# Autodesk Inventor assembly: Custom_Delta_Assembly
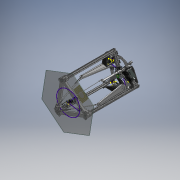
[picture p0: Inventor's stored thumbnail of the model, 180x180]
Saved by Autodesk Inventor 2019.4 (Build 234330000, 330)
## iProperties
Created: 2019-07-06
Part Number: Custom_Delta_Assembly
Document SubType Name: Assembly
Designer: Jorian Brusind
Author: Jorian Brusind
## Documents named in this file (20)
- C:\Users\Jorian Bruslind\Documents\GitHub\ECE44x_Senior_Design\Design files\Delta Robot Arm\Inventor Files\Custom_Delta\Custom_Delta_Assembly.iam
- C:\Users\Jorian Bruslind\Documents\GitHub\ECE44x_Senior_Design\Design files\Delta Robot Arm\Inventor Files\Custom_Delta\Stepper_Face.ipt
- C:\Users\Jorian Bruslind\Documents\GitHub\ECE44x_Senior_Design\Design files\Delta Robot Arm\Inventor Files\Custom_Delta\Delta_Arm.ipt
- C:\Users\Jorian Bruslind\Documents\GitHub\ECE44x_Senior_Design\Design files\Delta Robot Arm\Inventor Files\Custom_Delta\Delta_Top.ipt
- C:\Users\Jorian Bruslind\Documents\GitHub\ECE44x_Senior_Design\Design files\Delta Robot Arm\Inventor Files\McMaster Files\59935K140_METRIC BALL JOINT ROD END.ipt
- C:\Users\Jorian Bruslind\Documents\GitHub\ECE44x_Senior_Design\Design files\PetriFilm\PetriFilm.iam
- C:\Users\Jorian Bruslind\Documents\GitHub\ECE44x_Senior_Design\Design files\Delta Robot Arm\Inventor Files\McMaster Files\5537T501_ALUMINUM T-SLOTTED FRAMING EXTRUSION.ipt
- C:\Users\Jorian Bruslind\Documents\GitHub\ECE44x_Senior_Design\Design files\Delta Robot Arm\Inventor Files\McMaster Files\5537T518_T-SLOTTED FRAMING.ipt
- C:\Users\Jorian Bruslind\Documents\GitHub\ECE44x_Senior_Design\Design files\Delta Robot Arm\Inventor Files\McMaster Files\6In_ALUMINUM T-SLOTTED FRAMING EXTRUSION.ipt
- C:\Users\Jorian Bruslind\Documents\GitHub\ECE44x_Senior_Design\Design files\Delta Robot Arm\Inventor Files\Custom_Delta\Custom_Delta_End_Effector.ipt
- C:\Users\Jorian Bruslind\Documents\GitHub\ECE44x_Senior_Design\Design files\Delta Robot Arm\Inventor Files\Custom_Delta\80_20_Connector.ipt
- C:\Users\Jorian Bruslind\Documents\GitHub\ECE44x_Senior_Design\Design files\Delta Robot Arm\Inventor Files\Custom_Delta\NEMA17_Stepper_CL42H60.ipt
- C:\Users\Jorian Bruslind\Documents\GitHub\ECE44x_Senior_Design\Design files\Delta Robot Arm\Inventor Files\Stepper_Collar\products\12196\step\model.ipt
- C:\Users\Jorian Bruslind\Documents\GitHub\ECE44x_Senior_Design\Design files\Delta Robot Arm\Inventor Files\raspberry-pi-camera-module-v2-1.snapshot.3\RspCameraMia.iam
- C:\Users\Jorian Bruslind\Documents\GitHub\ECE44x_Senior_Design\Design files\Delta Robot Arm\Inventor Files\Custom_Delta\80_20_Connector_Bot.ipt
- C:\Users\Jorian Bruslind\Documents\GitHub\ECE44x_Senior_Design\Design files\Delta Robot Arm\Inventor Files\endstop-mechanical-limit-switch-on-pcb-1.snapshot.1\Switch.ipt
- C:\Users\Jorian Bruslind\Documents\GitHub\ECE44x_Senior_Design\Design files\Delta Robot Arm\Inventor Files\Metric bolt\Bolt M3 30mm.ipt
- C:\Users\Jorian Bruslind\Documents\GitHub\ECE44x_Senior_Design\Design files\Delta Robot Arm\Inventor Files\Custom_Delta\5mmSpacer.ipt
- C:\Users\Jorian Bruslind\Documents\GitHub\ECE44x_Senior_Design\Design files\Delta Robot Arm\Inventor Files\Custom_Delta\Bottom_Mount.ipt
- C:\Users\Jorian Bruslind\Documents\GitHub\ECE44x_Senior_Design\Design files\Delta Robot Arm\Inventor Files\McMaster Files\98861A050_LOW-STRENGTH STEEL THREADED ROD.ipt
## Components (60 placed, 19 different names)
1. Stepper_Face:1 — Mate:126, Flush:20, Flush:23, Mate:210, Mate:211, Mate:212, Mate:216
2. Delta_Arm:1 — Mate:145, Mate:146, Mate:214, Mate:215, Mate:254, Mate:360, Mate:361
3. Stepper_Face:2 — Mate:125, Flush:18, Flush:24, Mate:222, Mate:227, Mate:230, Mate:231
4. Delta_Arm:2 — Mate:151, Mate:152, Mate:220, Mate:221, Mate:253, Mate:321
5. Stepper_Face:3 — Mate:127, Flush:21, Flush:22, Mate:217, Mate:218, Mate:226, Mate:228
6. Delta_Arm:3 — Mate:224, Mate:225, Mate:229, Mate:333, Mate:341, Mate:345, Mate:346
7. Delta_Top:1 — Mate:103, Mate:105, Mate:106, Mate:107, Mate:109, Mate:110, Mate:111, Mate:112, Mate:113, Mate:189, Mate:190, Mate:191, Mate:192, Mate:238, Mate:240, Mate:241, Mate:243, Mate:244, Mate:246, Mate:368
8. 59935K140_METRIC BALL JOINT ROD END:2 — Mate:145, Mate:146
9. 59935K140_METRIC BALL JOINT ROD END:3 — Mate:151, Mate:152, Mate:270, Mate:271, Mate:374
10. PetriFilm:1 [sub-assembly]
11. 5537T518_T-SLOTTED FRAMING:1 — Mate:106, Mate:107, Mate:119, Flush:30
12. 5537T518_T-SLOTTED FRAMING:2 — Mate:103, Mate:105, Mate:118
13. 5537T518_T-SLOTTED FRAMING:3 — Mate:109, Mate:110, Mate:117
14. 6In_ALUMINUM T-SLOTTED FRAMING EXTRUSION:1 — Flush:5, Mate:121, Flush:6, Mate:126, Flush:20, Flush:23, Mate:188, Mate:235, Mate:247
15. 6In_ALUMINUM T-SLOTTED FRAMING EXTRUSION:2 — Flush:9, Flush:10, Mate:123, Mate:125, Flush:18, Flush:24, Mate:237
16. 6In_ALUMINUM T-SLOTTED FRAMING EXTRUSION:3 — Flush:7, Flush:8, Mate:122, Mate:127, Flush:21, Flush:22, Mate:233
17. 5537T501_ALUMINUM T-SLOTTED FRAMING EXTRUSION:1 — Mate:112, Mate:118, Flush:5, Mate:121, Flush:6, Mate:192, Mate:234, Flush:26, Mate:245, Mate:357, Mate:358
18. 5537T501_ALUMINUM T-SLOTTED FRAMING EXTRUSION:2 — Mate:111, Mate:119, Flush:7, Flush:8, Mate:122, Mate:190, Mate:232, Flush:25, Mate:239, Mate:355, Mate:359
19. 5537T501_ALUMINUM T-SLOTTED FRAMING EXTRUSION:3 — Mate:113, Mate:117, Flush:9, Flush:10, Mate:123, Mate:191, Mate:236, Flush:27, Mate:242, Mate:354, Mate:356
20. 80_20_Connector:1 — Mate:188, Mate:189, Mate:248, Mate:249, Mate:255, Mate:256, Mate:263, Mate:264, Mate:265, Mate:266, Mate:267
21. NEMA17_Stepper_CL42H60:1 — Mate:219, Mate:227, Mate:230, Mate:231
22. NEMA17_Stepper_CL42H60:2 — Mate:210, Mate:211, Mate:212, Mate:213
23. NEMA17_Stepper_CL42H60:3 — Mate:217, Mate:218, Mate:223, Mate:228
24. model:4 — Mate:223, Mate:224, Mate:225, Mate:226, Mate:229
25. model:5 — Mate:213, Mate:214, Mate:215, Mate:216, Mate:254
26. model:6 — Mate:219, Mate:220, Mate:221, Mate:222, Mate:253
27. 5537T518_T-SLOTTED FRAMING:4 — Mate:236, Mate:237, Flush:27
28. 5537T518_T-SLOTTED FRAMING:5 — Mate:232, Mate:233, Flush:25
29. 5537T518_T-SLOTTED FRAMING:6 — Mate:234, Mate:235, Flush:26
30. 5537T518_T-SLOTTED FRAMING:7 — Mate:238, Mate:239, Mate:240, Flush:28
31. 5537T518_T-SLOTTED FRAMING:8 — Mate:241, Mate:242, Mate:243
32. 5537T518_T-SLOTTED FRAMING:9 — Mate:244, Mate:245, Mate:246, Flush:29
33. RspCameraMia:1 [sub-assembly] — Mate:250, Mate:251, Mate:252
34. 80_20_Connector_Bot:1 — Mate:247, Mate:248, Mate:249, Mate:250, Mate:251, Mate:252
35. Switch:1 — Mate:255, Mate:256, Mate:263
36. Switch:2
37. Switch:3
38. 80_20_Connector:2 — Mate:264, Mate:265, Mate:266, Mate:268, Mate:269
39. 80_20_Connector:3 — Mate:267, Mate:268, Mate:269
40. Bolt M3 30mm:1 — Mate:270, Mate:271, Mate:299, Mate:320
41. 5mmSpacer:2 — Mate:299
42. 59935K140_METRIC BALL JOINT ROD END:17 — Mate:320, Mate:321, Mate:370, Mate:372
43. 59935K140_METRIC BALL JOINT ROD END:22 — Mate:333, Mate:346, Mate:380, Mate:382
44. 59935K140_METRIC BALL JOINT ROD END:23 — Mate:341, Mate:345, Mate:377, Mate:379
45. Bottom_Mount:1 — Mate:354, Mate:355, Flush:28
46. Bottom_Mount:3 — Mate:356, Mate:357, Flush:29
47. Bottom_Mount:4 — Mate:358, Mate:359, Flush:30
48. 59935K140_METRIC BALL JOINT ROD END:24 — Mate:360, Mate:361, Mate:385, Mate:386
49. 98861A050_LOW-STRENGTH STEEL THREADED ROD:2 — Mate:369, Mate:370, Mate:371, Mate:372
50. 98861A050_LOW-STRENGTH STEEL THREADED ROD:3 — Mate:376, Mate:377, Mate:378, Mate:379
51. 98861A050_LOW-STRENGTH STEEL THREADED ROD:4 — Mate:380, Mate:382, Mate:383
52. 98861A050_LOW-STRENGTH STEEL THREADED ROD:5 — Mate:373, Mate:374, Mate:375
53. 98861A050_LOW-STRENGTH STEEL THREADED ROD:6 — Mate:384, Mate:385, Mate:386, Mate:387
54. 59935K140_METRIC BALL JOINT ROD END:25 — Mate:364, Mate:376, Mate:378
55. 59935K140_METRIC BALL JOINT ROD END:26 — Mate:363, Mate:369, Mate:371
56. 59935K140_METRIC BALL JOINT ROD END:27 — Mate:366, Mate:384, Mate:387
57. 59935K140_METRIC BALL JOINT ROD END:28 — Mate:362, Mate:373, Mate:375
58. 59935K140_METRIC BALL JOINT ROD END:29 — Mate:367
59. 59935K140_METRIC BALL JOINT ROD END:30 — Mate:365, Mate:383
60. Custom_Delta_End_Effector:1 — Mate:362, Mate:363, Mate:364, Mate:365, Mate:366, Mate:367, Mate:368
## Relationships (141: Mate 123, Flush 18)
- Mate:103: Delta_Top:1 ↔ 5537T518_T-SLOTTED FRAMING:2
- Mate:105: Delta_Top:1 ↔ 5537T518_T-SLOTTED FRAMING:2
- Mate:106: Delta_Top:1 ↔ 5537T518_T-SLOTTED FRAMING:1
- Mate:107: Delta_Top:1 ↔ 5537T518_T-SLOTTED FRAMING:1
- Mate:109: Delta_Top:1 ↔ 5537T518_T-SLOTTED FRAMING:3
- Mate:110: Delta_Top:1 ↔ 5537T518_T-SLOTTED FRAMING:3
- Mate:111: Delta_Top:1 ↔ 5537T501_ALUMINUM T-SLOTTED FRAMING EXTRUSION:2
- Mate:112: Delta_Top:1 ↔ 5537T501_ALUMINUM T-SLOTTED FRAMING EXTRUSION:1
- Mate:113: Delta_Top:1 ↔ 5537T501_ALUMINUM T-SLOTTED FRAMING EXTRUSION:3
- Mate:117: 5537T518_T-SLOTTED FRAMING:3 ↔ 5537T501_ALUMINUM T-SLOTTED FRAMING EXTRUSION:3
- Mate:118: 5537T518_T-SLOTTED FRAMING:2 ↔ 5537T501_ALUMINUM T-SLOTTED FRAMING EXTRUSION:1
- Mate:119: 5537T518_T-SLOTTED FRAMING:1 ↔ 5537T501_ALUMINUM T-SLOTTED FRAMING EXTRUSION:2
- Flush:5: 6In_ALUMINUM T-SLOTTED FRAMING EXTRUSION:1 ↔ 5537T501_ALUMINUM T-SLOTTED FRAMING EXTRUSION:1
- Mate:121: 6In_ALUMINUM T-SLOTTED FRAMING EXTRUSION:1 ↔ 5537T501_ALUMINUM T-SLOTTED FRAMING EXTRUSION:1
- Flush:6: 6In_ALUMINUM T-SLOTTED FRAMING EXTRUSION:1 ↔ 5537T501_ALUMINUM T-SLOTTED FRAMING EXTRUSION:1
- Flush:7: 6In_ALUMINUM T-SLOTTED FRAMING EXTRUSION:3 ↔ 5537T501_ALUMINUM T-SLOTTED FRAMING EXTRUSION:2
- Flush:8: 6In_ALUMINUM T-SLOTTED FRAMING EXTRUSION:3 ↔ 5537T501_ALUMINUM T-SLOTTED FRAMING EXTRUSION:2
- Mate:122: 6In_ALUMINUM T-SLOTTED FRAMING EXTRUSION:3 ↔ 5537T501_ALUMINUM T-SLOTTED FRAMING EXTRUSION:2
- Flush:9: 6In_ALUMINUM T-SLOTTED FRAMING EXTRUSION:2 ↔ 5537T501_ALUMINUM T-SLOTTED FRAMING EXTRUSION:3
- Flush:10: 6In_ALUMINUM T-SLOTTED FRAMING EXTRUSION:2 ↔ 5537T501_ALUMINUM T-SLOTTED FRAMING EXTRUSION:3
- Mate:123: 6In_ALUMINUM T-SLOTTED FRAMING EXTRUSION:2 ↔ 5537T501_ALUMINUM T-SLOTTED FRAMING EXTRUSION:3
- Mate:125: Stepper_Face:2 ↔ 6In_ALUMINUM T-SLOTTED FRAMING EXTRUSION:2
- Mate:126: Stepper_Face:1 ↔ 6In_ALUMINUM T-SLOTTED FRAMING EXTRUSION:1
- Mate:127: Stepper_Face:3 ↔ 6In_ALUMINUM T-SLOTTED FRAMING EXTRUSION:3
- Mate:145: Delta_Arm:1 ↔ 59935K140_METRIC BALL JOINT ROD END:2
- Mate:146 (2.5 mm): Delta_Arm:1 ↔ 59935K140_METRIC BALL JOINT ROD END:2
- Mate:151: Delta_Arm:2 ↔ 59935K140_METRIC BALL JOINT ROD END:3
- Mate:152 (2.5 mm): Delta_Arm:2 ↔ 59935K140_METRIC BALL JOINT ROD END:3
- Flush:18: Stepper_Face:2 ↔ 6In_ALUMINUM T-SLOTTED FRAMING EXTRUSION:2
- Flush:20: Stepper_Face:1 ↔ 6In_ALUMINUM T-SLOTTED FRAMING EXTRUSION:1
- Flush:21: Stepper_Face:3 ↔ 6In_ALUMINUM T-SLOTTED FRAMING EXTRUSION:3
- Flush:22 (112.406 mm): Stepper_Face:3 ↔ 6In_ALUMINUM T-SLOTTED FRAMING EXTRUSION:3
- Flush:23 (112.206 mm): Stepper_Face:1 ↔ 6In_ALUMINUM T-SLOTTED FRAMING EXTRUSION:1
- Flush:24 (112.406 mm): Stepper_Face:2 ↔ 6In_ALUMINUM T-SLOTTED FRAMING EXTRUSION:2
- Mate:188: 6In_ALUMINUM T-SLOTTED FRAMING EXTRUSION:1 ↔ 80_20_Connector:1
- Mate:189: Delta_Top:1 ↔ 80_20_Connector:1
- Mate:190: Delta_Top:1 ↔ 5537T501_ALUMINUM T-SLOTTED FRAMING EXTRUSION:2
- Mate:191: Delta_Top:1 ↔ 5537T501_ALUMINUM T-SLOTTED FRAMING EXTRUSION:3
- Mate:192: Delta_Top:1 ↔ 5537T501_ALUMINUM T-SLOTTED FRAMING EXTRUSION:1
- Mate:210: Stepper_Face:1 ↔ NEMA17_Stepper_CL42H60:2
- Mate:211: Stepper_Face:1 ↔ NEMA17_Stepper_CL42H60:2
- Mate:212: Stepper_Face:1 ↔ NEMA17_Stepper_CL42H60:2
- Mate:213: NEMA17_Stepper_CL42H60:2 ↔ model:5
- Mate:214: Delta_Arm:1 ↔ model:5
- Mate:215: Delta_Arm:1 ↔ model:5
- Mate:216: Stepper_Face:1 ↔ model:5
- Mate:217: Stepper_Face:3 ↔ NEMA17_Stepper_CL42H60:3
- Mate:218: Stepper_Face:3 ↔ NEMA17_Stepper_CL42H60:3
- Mate:219: NEMA17_Stepper_CL42H60:1 ↔ model:6
- Mate:220: Delta_Arm:2 ↔ model:6
- Mate:221: Delta_Arm:2 ↔ model:6
- Mate:222: Stepper_Face:2 ↔ model:6
- Mate:223: NEMA17_Stepper_CL42H60:3 ↔ model:4
- Mate:224: Delta_Arm:3 ↔ model:4
- Mate:225: Delta_Arm:3 ↔ model:4
- Mate:226: Stepper_Face:3 ↔ model:4
- Mate:227: Stepper_Face:2 ↔ NEMA17_Stepper_CL42H60:1
- Mate:228: Stepper_Face:3 ↔ NEMA17_Stepper_CL42H60:3
- Mate:229: Delta_Arm:3 ↔ model:4
- Mate:230: Stepper_Face:2 ↔ NEMA17_Stepper_CL42H60:1
- Mate:231: Stepper_Face:2 ↔ NEMA17_Stepper_CL42H60:1
- Mate:232: 5537T501_ALUMINUM T-SLOTTED FRAMING EXTRUSION:2 ↔ 5537T518_T-SLOTTED FRAMING:5
- Mate:233: 6In_ALUMINUM T-SLOTTED FRAMING EXTRUSION:3 ↔ 5537T518_T-SLOTTED FRAMING:5
- Flush:25: 5537T501_ALUMINUM T-SLOTTED FRAMING EXTRUSION:2 ↔ 5537T518_T-SLOTTED FRAMING:5
- Mate:234: 5537T501_ALUMINUM T-SLOTTED FRAMING EXTRUSION:1 ↔ 5537T518_T-SLOTTED FRAMING:6
- Mate:235: 6In_ALUMINUM T-SLOTTED FRAMING EXTRUSION:1 ↔ 5537T518_T-SLOTTED FRAMING:6
- Flush:26: 5537T501_ALUMINUM T-SLOTTED FRAMING EXTRUSION:1 ↔ 5537T518_T-SLOTTED FRAMING:6
- Mate:236: 5537T501_ALUMINUM T-SLOTTED FRAMING EXTRUSION:3 ↔ 5537T518_T-SLOTTED FRAMING:4
- Mate:237: 6In_ALUMINUM T-SLOTTED FRAMING EXTRUSION:2 ↔ 5537T518_T-SLOTTED FRAMING:4
- Flush:27: 5537T501_ALUMINUM T-SLOTTED FRAMING EXTRUSION:3 ↔ 5537T518_T-SLOTTED FRAMING:4
- Mate:238: Delta_Top:1 ↔ 5537T518_T-SLOTTED FRAMING:7
- Mate:239: 5537T501_ALUMINUM T-SLOTTED FRAMING EXTRUSION:2 ↔ 5537T518_T-SLOTTED FRAMING:7
- Mate:240: Delta_Top:1 ↔ 5537T518_T-SLOTTED FRAMING:7
- Mate:241: Delta_Top:1 ↔ 5537T518_T-SLOTTED FRAMING:8
- Mate:242: 5537T501_ALUMINUM T-SLOTTED FRAMING EXTRUSION:3 ↔ 5537T518_T-SLOTTED FRAMING:8
- Mate:243: Delta_Top:1 ↔ 5537T518_T-SLOTTED FRAMING:8
- Mate:244: Delta_Top:1 ↔ 5537T518_T-SLOTTED FRAMING:9
- Mate:245: 5537T501_ALUMINUM T-SLOTTED FRAMING EXTRUSION:1 ↔ 5537T518_T-SLOTTED FRAMING:9
- Mate:246: Delta_Top:1 ↔ 5537T518_T-SLOTTED FRAMING:9
- Mate:247: 6In_ALUMINUM T-SLOTTED FRAMING EXTRUSION:1 ↔ 80_20_Connector_Bot:1
- Mate:248: 80_20_Connector:1 ↔ 80_20_Connector_Bot:1
- Mate:249: 80_20_Connector:1 ↔ 80_20_Connector_Bot:1
- Mate:250: RspCameraMia:1 ↔ 80_20_Connector_Bot:1
- Mate:251: RspCameraMia:1 ↔ 80_20_Connector_Bot:1
- Mate:252: RspCameraMia:1 ↔ 80_20_Connector_Bot:1
- Mate:253: Delta_Arm:2 ↔ model:6
- Mate:254: Delta_Arm:1 ↔ model:5
- Mate:255: 80_20_Connector:1 ↔ Switch:1
- Mate:256: 80_20_Connector:1 ↔ Switch:1
- Mate:263: 80_20_Connector:1 ↔ Switch:1
- Mate:264: 80_20_Connector:1 ↔ 80_20_Connector:2
- Mate:265: 80_20_Connector:1 ↔ 80_20_Connector:2
- Mate:266: 80_20_Connector:1 ↔ 80_20_Connector:2
- Mate:267: 80_20_Connector:1 ↔ 80_20_Connector:3
- Mate:268: 80_20_Connector:2 ↔ 80_20_Connector:3
- Mate:269: 80_20_Connector:2 ↔ 80_20_Connector:3
- Mate:270: 59935K140_METRIC BALL JOINT ROD END:3 ↔ Bolt M3 30mm:1
- Mate:271: 59935K140_METRIC BALL JOINT ROD END:3 ↔ Bolt M3 30mm:1
- Mate:299: Bolt M3 30mm:1 ↔ 5mmSpacer:2
- Mate:320: Bolt M3 30mm:1 ↔ 59935K140_METRIC BALL JOINT ROD END:17
- Mate:321 (2.5 mm): Delta_Arm:2 ↔ 59935K140_METRIC BALL JOINT ROD END:17
- Mate:333: Delta_Arm:3 ↔ 59935K140_METRIC BALL JOINT ROD END:22
- Mate:341: Delta_Arm:3 ↔ 59935K140_METRIC BALL JOINT ROD END:23
- Mate:345 (2.5 mm): Delta_Arm:3 ↔ 59935K140_METRIC BALL JOINT ROD END:23
- Mate:346 (2.5 mm): Delta_Arm:3 ↔ 59935K140_METRIC BALL JOINT ROD END:22
- Mate:354: 5537T501_ALUMINUM T-SLOTTED FRAMING EXTRUSION:3 ↔ Bottom_Mount:1
- Mate:355: 5537T501_ALUMINUM T-SLOTTED FRAMING EXTRUSION:2 ↔ Bottom_Mount:1
- Flush:28: 5537T518_T-SLOTTED FRAMING:7 ↔ Bottom_Mount:1
- Mate:356: 5537T501_ALUMINUM T-SLOTTED FRAMING EXTRUSION:3 ↔ Bottom_Mount:3
- Mate:357: 5537T501_ALUMINUM T-SLOTTED FRAMING EXTRUSION:1 ↔ Bottom_Mount:3
- Flush:29: 5537T518_T-SLOTTED FRAMING:9 ↔ Bottom_Mount:3
- Mate:358: 5537T501_ALUMINUM T-SLOTTED FRAMING EXTRUSION:1 ↔ Bottom_Mount:4
- Mate:359: 5537T501_ALUMINUM T-SLOTTED FRAMING EXTRUSION:2 ↔ Bottom_Mount:4
- Flush:30: 5537T518_T-SLOTTED FRAMING:1 ↔ Bottom_Mount:4
- Mate:360: Delta_Arm:1 ↔ 59935K140_METRIC BALL JOINT ROD END:24
- Mate:361 (2.5 mm): Delta_Arm:1 ↔ 59935K140_METRIC BALL JOINT ROD END:24
- Mate:362: 59935K140_METRIC BALL JOINT ROD END:28 ↔ Custom_Delta_End_Effector:1
- Mate:363: 59935K140_METRIC BALL JOINT ROD END:26 ↔ Custom_Delta_End_Effector:1
- Mate:364: 59935K140_METRIC BALL JOINT ROD END:25 ↔ Custom_Delta_End_Effector:1
- Mate:365: 59935K140_METRIC BALL JOINT ROD END:30 ↔ Custom_Delta_End_Effector:1
- Mate:366: 59935K140_METRIC BALL JOINT ROD END:27 ↔ Custom_Delta_End_Effector:1
- Mate:367: 59935K140_METRIC BALL JOINT ROD END:29 ↔ Custom_Delta_End_Effector:1
- Mate:368: Delta_Top:1 ↔ Custom_Delta_End_Effector:1
- Mate:369: 98861A050_LOW-STRENGTH STEEL THREADED ROD:2 ↔ 59935K140_METRIC BALL JOINT ROD END:26
- Mate:370: 59935K140_METRIC BALL JOINT ROD END:17 ↔ 98861A050_LOW-STRENGTH STEEL THREADED ROD:2
- Mate:371: 98861A050_LOW-STRENGTH STEEL THREADED ROD:2 ↔ 59935K140_METRIC BALL JOINT ROD END:26
- Mate:372: 59935K140_METRIC BALL JOINT ROD END:17 ↔ 98861A050_LOW-STRENGTH STEEL THREADED ROD:2
- Mate:373: 98861A050_LOW-STRENGTH STEEL THREADED ROD:5 ↔ 59935K140_METRIC BALL JOINT ROD END:28
- Mate:374: 59935K140_METRIC BALL JOINT ROD END:3 ↔ 98861A050_LOW-STRENGTH STEEL THREADED ROD:5
- Mate:375: 98861A050_LOW-STRENGTH STEEL THREADED ROD:5 ↔ 59935K140_METRIC BALL JOINT ROD END:28
- Mate:376: 98861A050_LOW-STRENGTH STEEL THREADED ROD:3 ↔ 59935K140_METRIC BALL JOINT ROD END:25
- Mate:377: 59935K140_METRIC BALL JOINT ROD END:23 ↔ 98861A050_LOW-STRENGTH STEEL THREADED ROD:3
- Mate:378: 98861A050_LOW-STRENGTH STEEL THREADED ROD:3 ↔ 59935K140_METRIC BALL JOINT ROD END:25
- Mate:379: 59935K140_METRIC BALL JOINT ROD END:23 ↔ 98861A050_LOW-STRENGTH STEEL THREADED ROD:3
- Mate:380: 59935K140_METRIC BALL JOINT ROD END:22 ↔ 98861A050_LOW-STRENGTH STEEL THREADED ROD:4
- Mate:382: 59935K140_METRIC BALL JOINT ROD END:22 ↔ 98861A050_LOW-STRENGTH STEEL THREADED ROD:4
- Mate:383: 98861A050_LOW-STRENGTH STEEL THREADED ROD:4 ↔ 59935K140_METRIC BALL JOINT ROD END:30
- Mate:384: 98861A050_LOW-STRENGTH STEEL THREADED ROD:6 ↔ 59935K140_METRIC BALL JOINT ROD END:27
- Mate:385: 59935K140_METRIC BALL JOINT ROD END:24 ↔ 98861A050_LOW-STRENGTH STEEL THREADED ROD:6
- Mate:386: 59935K140_METRIC BALL JOINT ROD END:24 ↔ 98861A050_LOW-STRENGTH STEEL THREADED ROD:6
- Mate:387: 98861A050_LOW-STRENGTH STEEL THREADED ROD:6 ↔ 59935K140_METRIC BALL JOINT ROD END:27
